# Autodesk Inventor assembly: mppcInterface
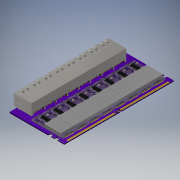
[picture p0: Inventor's stored thumbnail of the model, 180x180]
Saved by Autodesk Inventor 2016 (Build 200138000, 138)
## iProperties
Created: 2016-04-06
Part Number: mppcInterface
Document SubType Name: Assembly
Designer: sawai
Author: sawai
## Documents named in this file (4)
- C:\Users\Jonathan\Documents\Projects\mppcInterface\mppcInterface\cad\mppcInterface.iam
- C:\Users\Jonathan\Documents\Projects\mppcInterface\mppcInterface\cad\mppcInterfacePcb.ipt
- C:\Users\Jonathan\Documents\Projects\mppcInterface\mppcInterface\cad\dependency\mppcHighVoltage\cad\highVoltageMppcBoard.iam
- C:\Users\Jonathan\Documents\Projects\mppcInterface\mppcInterface\cad\connector\SS-668808S-A-PG4-AC.ipt
## Components (10 placed, 3 different names)
1. mppcInterfacePcb:1 — Mate:1, Angle:1, Angle:2, Mate:2
2. SS-668808S-A-PG4-AC:1 — Angle:2, Mate:2
3. highVoltageMppcBoard:1 [sub-assembly] — Mate:1, Angle:1
4. highVoltageMppcBoard:2 [sub-assembly]
5. highVoltageMppcBoard:3 [sub-assembly]
6. highVoltageMppcBoard:4 [sub-assembly]
7. highVoltageMppcBoard:5 [sub-assembly]
8. highVoltageMppcBoard:6 [sub-assembly]
9. highVoltageMppcBoard:7 [sub-assembly]
10. highVoltageMppcBoard:8 [sub-assembly]
## Component patterns: (8 elements, first: highVoltageMppcBoard:1)
## Relationships (4: Mate 2, Angle 2)
- Mate:1: mppcInterfacePcb:1 ↔ highVoltageMppcBoard:1
- Angle:1 (180 deg): mppcInterfacePcb:1 ↔ highVoltageMppcBoard:1
- Angle:2 (0 deg): mppcInterfacePcb:1 ↔ SS-668808S-A-PG4-AC:1
- Mate:2: mppcInterfacePcb:1 ↔ SS-668808S-A-PG4-AC:1
